# Autodesk Inventor assembly: Elevator Mock-up
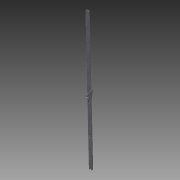
[picture p0: Inventor's stored thumbnail of the model, 180x180]
Saved by Autodesk Inventor 2015 (Build 190159000, 159)
## iProperties
Created: 2015-01-27
Part Number: Elevator Mock-up
Document SubType Name: Assembly
Designer: chapale16
Author: chapale16
## Documents named in this file (7)
- \\lhssvr02\Homedirs\Robotics Club\CAD Model 2015\Elevator parts\Elevator Mock-up.iam
- \\lhssvr02\Homedirs\Robotics Club\CAD Model 2015\Parts Folder\Stock\c hannel.ipt
- \\lhssvr02\Homedirs\Robotics Club\CAD Model 2015\Box Beam Drive Base\Elevator Latch.ipt
- \\lhssvr02\Homedirs\Robotics Club\CAD Model 2015\Elevator parts\mounting bracket.ipt
- \\lhssvr02\Homedirs\Robotics Club\CAD Model 2015\Elevator parts\Pneumatic piston.iam
- C:\Users\chapale16\Documents\D-14043.ipt
- C:\Users\chapale16\Documents\D-12304.ipt
## Components (7 placed, 6 different names)
1. c hannel:1 — Mate:3, Mate:4, Mate:7, Angle:1, Mate:8, Mate:17
2. Elevator Latch:1 — Mate:3, Mate:4, Mate:14
3. mounting bracket:1 — Mate:7, Angle:1, Mate:8, Mate:9, Mate:13
4. Pneumatic piston:2 [sub-assembly] — Mate:9, Mate:12, Angle:2, Mate:13, Mate:15, Mate:16
5. D-14043:1 — Flush:1, Mate:11, Mate:12, Angle:2
6. D-12304:1 — Flush:1, Mate:11, Mate:14
7. mounting bracket:2 — Mate:15, Mate:16, Mate:17
## Relationships (15: Mate 12, Angle 2, Flush 1)
- Mate:3: c hannel:1 ↔ Elevator Latch:1
- Mate:4: c hannel:1 ↔ Elevator Latch:1
- Mate:7: c hannel:1 ↔ mounting bracket:1
- Angle:1 (0 deg): c hannel:1 ↔ mounting bracket:1
- Mate:8: c hannel:1 ↔ mounting bracket:1
- Mate:9: mounting bracket:1 ↔ Pneumatic piston:2
- Flush:1: D-14043:1 ↔ D-12304:1
- Mate:11: D-14043:1 ↔ D-12304:1
- Mate:12: Pneumatic piston:2 ↔ D-14043:1
- Angle:2 (0 deg): Pneumatic piston:2 ↔ D-14043:1
- Mate:13: mounting bracket:1 ↔ Pneumatic piston:2
- Mate:14: Elevator Latch:1 ↔ D-12304:1
- Mate:15: Pneumatic piston:2 ↔ mounting bracket:2
- Mate:16: Pneumatic piston:2 ↔ mounting bracket:2
- Mate:17: c hannel:1 ↔ mounting bracket:2
